# Autodesk Inventor assembly: Assembly
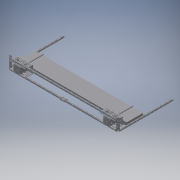
[picture p0: Inventor's stored thumbnail of the model, 180x180]
Saved by Autodesk Inventor 2019 (Build 230136000, 136)
## iProperties
Created: 2022-09-04
Part Number: Assembly
Document SubType Name: Assembly
Designer: Garrett Raker
Author: Garrett Raker
## Documents named in this file (6)
- F:\College Stuff\ATMAE Robotics\Pill Dispenser Robot\Assembly.iam
- F:\College Stuff\ATMAE Robotics\Pill Dispenser Robot\Base Structure\Base Assembly.iam
- F:\College Stuff\ATMAE Robotics\Pill Dispenser Robot\Base Structure\1308 Series Lightweight Set Screw Hub (4mm Bore).iam
- F:\College Stuff\ATMAE Robotics\Pill Dispenser Robot\Conveyor System\Conveyor System Assembly.iam
- F:\College Stuff\ATMAE Robotics\Pill Dispenser Robot\Conveyor System\Conveyor System Assembly_MIR.iam
- F:\College Stuff\ATMAE Robotics\Pill Dispenser Robot\Metal Platform.ipt
## Components (5 placed, 5 different names)
1. Base Assembly:1 [sub-assembly] — Mate:1, Angle:1, Flush:1, Angle:2, Mate:26, Mate:27, Mate:28, Mate:29, Mate:30, Mate:31, Mate:32, Flush:2
2. 1308 Series Lightweight Set Screw Hub (4mm Bore):1 [sub-assembly]
3. Conveyor System Assembly:1 [sub-assembly] — Mate:29, Mate:30, Mate:31, Flush:3
4. Conveyor System Assembly_MIR:1 [sub-assembly]
5. Metal Platform:1 — Mate:32, Flush:2, Flush:3
## Relationships (15: Mate 10, Flush 3, Angle 2)
- Mate:1: Base Assembly:1
- Mate:2
- Angle:1 (90 deg): Base Assembly:1
- Flush:1 (6.35 mm): Base Assembly:1
- Mate:5
- Angle:2 (90 deg): Base Assembly:1
- Mate:26: Base Assembly:1
- Mate:27: Base Assembly:1
- Mate:28: Base Assembly:1
- Mate:29: Base Assembly:1 ↔ Conveyor System Assembly:1
- Mate:30: Base Assembly:1 ↔ Conveyor System Assembly:1
- Mate:31: Base Assembly:1 ↔ Conveyor System Assembly:1
- Mate:32: Base Assembly:1 ↔ Metal Platform:1
- Flush:2: Base Assembly:1 ↔ Metal Platform:1
- Flush:3: Conveyor System Assembly:1 ↔ Metal Platform:1
